# Autodesk Inventor assembly: omni_platforma_plata
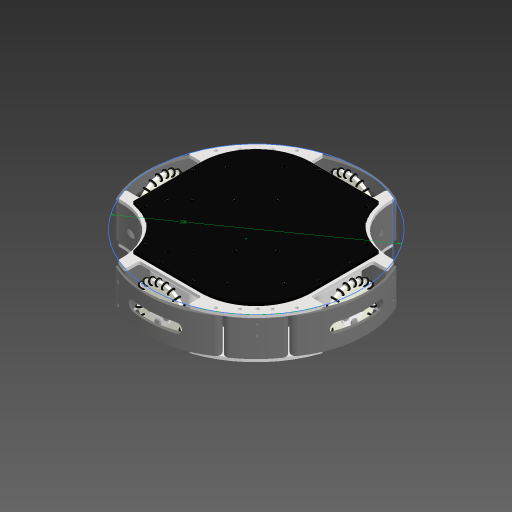
[picture p0: Inventor's stored thumbnail of the model, 512x512]
Saved by Autodesk Inventor 2023 (Build 270158000, 158)
## iProperties
Created: 2025-07-17
Part Number: omni_platforma_plata
Document SubType Name: Assembly
Designer: daa
Author: daa
## Documents named in this file (3)
- C:\Users\daa\Documents\DASH_V2\omni_platforma\omni_platforma_plata.iam
- C:\Users\daa\Documents\DASH_V2\omni_platforma\omni_platforma.iam
- C:\Users\daa\Documents\DASH_V2\omni_platforma\plat.ipt
## Components (2 placed, 2 different names)
1. omni_platforma:1 [sub-assembly] — Совмещение:1, С поворотом:1
2. plat:1 — Совмещение:1, С поворотом:1
## Relationships (2: Mate 1, RevoluteJoint 1)
- Совмещение:1 [Mate] (3 mm): omni_platforma:1 ↔ plat:1
- С поворотом:1 [RevoluteJoint] (-3 mm): omni_platforma:1 ↔ plat:1
